# Autodesk Inventor assembly: MaxonEC45-50W-MILE-Machined-with-gear
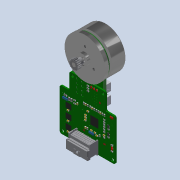
[picture p0: Inventor's stored thumbnail of the model, 180x180]
Saved by Autodesk Inventor 2020.4 (Build 244396000, 396)
## iProperties
Created: 2015-08-10
Part Number: MaxonEC45-50W-MILE-Machined-with-gear
Document SubType Name: Assembly
Designer: ryll
Author: ryll
## Documents named in this file (6)
- G:\Meu Drive\RobôCIn\Mecânica\SSL\2021\Inventor\first_floor\Motor\MaxonEC45-50W-MILE-Machined-with-gear.iam
- G:\Meu Drive\RobôCIn\Mecânica\SSL\2021\Inventor\first_floor\Motor\MaxonEC45-50W-MILE.ipt
- G:\Meu Drive\RobôCIn\Mecânica\SSL\2021\Inventor\first_floor\Motor\IDC Stecker 10pol.ipt
- G:\Meu Drive\RobôCIn\Mecânica\SSL\2021\Inventor\first_floor\Motor\Molex MiniFit 8pol.ipt
- G:\Meu Drive\RobôCIn\Mecânica\SSL\2021\Inventor\first_floor\Motor\gear_z18_21101800(modified).ipt
- G:\Meu Drive\RobôCIn\Mecânica\SSL\2021\Inventor\first_floor\Components\MotorBoard\MOTORBOARD_V1.0.IAM
## Components (5 placed, 5 different names)
1. MaxonEC45-50W-MILE:1 — Passend:1, Passend:2, Fluchtend:1, Fluchtend:2, Fluchtend:3, Fluchtend:4, Mate:3, Mate:4, Mate:5, Mate:6, Mate:7
2. IDC Stecker 10pol:1 — Passend:2, Fluchtend:1, Fluchtend:2
3. Molex MiniFit 8pol:1 — Passend:1, Fluchtend:3, Fluchtend:4
4. Ritzel z=18:1 — Mate:3, Mate:4
5. MOTORBOARD_V1.0:1 [sub-assembly] — Mate:5, Mate:6, Mate:7
## Relationships (11: Mate 7, Flush 4)
- Passend:1 [Mate]: MaxonEC45-50W-MILE:1 ↔ Molex MiniFit 8pol:1
- Passend:2 [Mate]: MaxonEC45-50W-MILE:1 ↔ IDC Stecker 10pol:1
- Fluchtend:1 [Flush] (2 mm): MaxonEC45-50W-MILE:1 ↔ IDC Stecker 10pol:1
- Fluchtend:2 [Flush] (4 mm): MaxonEC45-50W-MILE:1 ↔ IDC Stecker 10pol:1
- Fluchtend:3 [Flush] (4 mm): MaxonEC45-50W-MILE:1 ↔ Molex MiniFit 8pol:1
- Fluchtend:4 [Flush] (4 mm): MaxonEC45-50W-MILE:1 ↔ Molex MiniFit 8pol:1
- Mate:3: MaxonEC45-50W-MILE:1 ↔ Ritzel z=18:1
- Mate:4 (1 mm): MaxonEC45-50W-MILE:1 ↔ Ritzel z=18:1
- Mate:5: MaxonEC45-50W-MILE:1 ↔ MOTORBOARD_V1.0:1
- Mate:6 (-22.5 mm): MaxonEC45-50W-MILE:1 ↔ MOTORBOARD_V1.0:1
- Mate:7 (-37.25 mm): MaxonEC45-50W-MILE:1 ↔ MOTORBOARD_V1.0:1
